# Autodesk Inventor assembly: motor_set
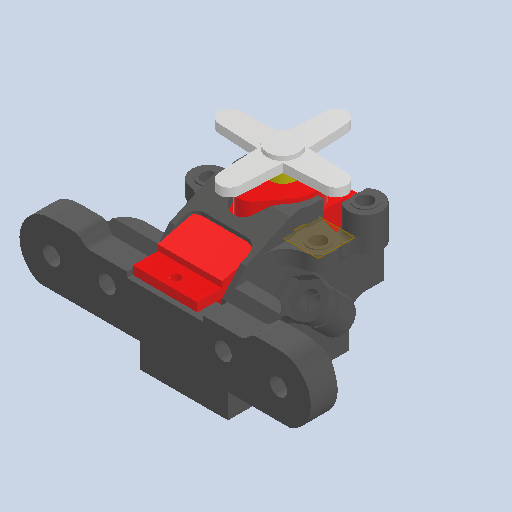
[picture p0: Inventor's stored thumbnail of the model, 512x512]
Saved by Autodesk Inventor 2024.1 (Build 281209000, 209)
## iProperties
Created: 2024-12-19
Part Number: motor_set
Document SubType Name: Assembly
Designer: hibik
Author: hibik
## Documents named in this file (4)
- C:\Users\hibik\Documents\Robomech\RESCUE\ORCA\hard\omni_wheel\motor_set.iam
- C:\Users\hibik\Documents\Robomech\RESCUE\ORCA\hard\std_parts\FT90MR.ipt
- C:\Users\hibik\Documents\Robomech\RESCUE\ORCA\hard\omni_wheel\motor_cover_under.ipt
- C:\Users\hibik\Documents\Robomech\RESCUE\ORCA\hard\omni_wheel\motor_cover_upper.ipt
## Components (3 placed, 3 different names)
1. FT90MR:1 — メイト:1, メイト:2, メイト:3, メイト:4, メイト:5, メイト:6
2. motor_cover_under:1 — メイト:4, メイト:5, メイト:6, フラッシュ:2, フラッシュ:3
3. motor_cover_upper:1 — メイト:1, メイト:2, メイト:3, フラッシュ:2, フラッシュ:3
## Relationships (8: Mate 6, Flush 2)
- メイト:1 [Mate] (0.1 mm): FT90MR:1 ↔ motor_cover_upper:1
- メイト:2 [Mate]: FT90MR:1 ↔ motor_cover_upper:1
- メイト:3 [Mate] (0.1 mm): FT90MR:1 ↔ motor_cover_upper:1
- メイト:4 [Mate] (0.1 mm): FT90MR:1 ↔ motor_cover_under:1
- メイト:5 [Mate] (0.1 mm): FT90MR:1 ↔ motor_cover_under:1
- メイト:6 [Mate] (0.1 mm): FT90MR:1 ↔ motor_cover_under:1
- フラッシュ:2 [Flush] (0.5 mm): motor_cover_under:1 ↔ motor_cover_upper:1
- フラッシュ:3 [Flush]: motor_cover_under:1 ↔ motor_cover_upper:1
